# Autodesk Inventor assembly: multiples_bouteilles
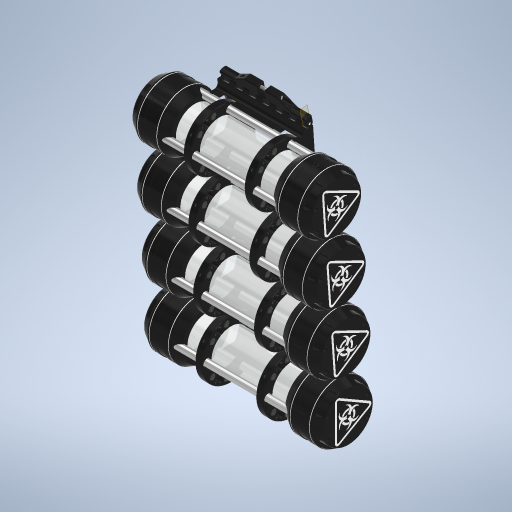
[picture p0: Inventor's stored thumbnail of the model, 512x512]
Saved by Autodesk Inventor 2024.2 (Build 282272000, 272)
## iProperties
Created: 2024-10-04
Part Number: multiples_bouteilles
Document SubType Name: Assembly
Designer: Sebastien
Author: Sebastien
## Documents named in this file (5)
- D:\Projets\BottleLeds\CAD\multiples_bouteilles.iam
- D:\Projets\BottleLeds\CAD\EG.iam
- D:\Projets\BottleLeds\CAD\adaptateur_sangle.ipt
- C:\Users\Sebastien\Documents\Inventor\Content Center Files\R2024\fr-FR\ISO 4762(2)\ISO 4762 - M4 x 40ISO.ipt
- D:\Projets\BottleLeds\CAD\adaptateur_sangle_large.ipt
## Components (8 placed, 4 different names)
1. EG:1 [sub-assembly] — Placage:1, Affleurement:1, Placage:2, Placage:3, Placage:10
2. adaptateur_sangle:1 — Affleurement:1, Placage:2, Logement:1
3. ISO 4762 M4 x 40:1 — Logement:1
4. adaptateur_sangle_large:2 — Logement:2, Placage:6, Placage:7
5. ISO 4762 M4 x 40:2 — Logement:2
6. EG:2 [sub-assembly] — Placage:3, Placage:4, Placage:9, Placage:10
7. EG:3 [sub-assembly] — Placage:4, Placage:5, Placage:8, Placage:9
8. EG:4 [sub-assembly] — Placage:5, Placage:6, Placage:7, Placage:8
## Relationships (13: Mate 10, Insert 2, Flush 1)
- Placage:1 [Mate]: EG:1
- Affleurement:1 [Flush]: EG:1 ↔ adaptateur_sangle:1
- Placage:2 [Mate]: EG:1 ↔ adaptateur_sangle:1
- Logement:1 [Insert]: adaptateur_sangle:1 ↔ ISO 4762 M4 x 40:1
- Logement:2 [Insert]: adaptateur_sangle_large:2 ↔ ISO 4762 M4 x 40:2
- Placage:3 [Mate]: EG:1 ↔ EG:2
- Placage:4 [Mate]: EG:2 ↔ EG:3
- Placage:5 [Mate]: EG:3 ↔ EG:4
- Placage:6 [Mate]: adaptateur_sangle_large:2 ↔ EG:4
- Placage:7 [Mate]: adaptateur_sangle_large:2 ↔ EG:4
- Placage:8 [Mate]: EG:3 ↔ EG:4
- Placage:9 [Mate]: EG:2 ↔ EG:3
- Placage:10 [Mate]: EG:1 ↔ EG:2
## Named parameters: d19_d16 = 0 mm, d20_d17 = 0 mm, d21_d18 = 0 mm
